# Autodesk Inventor assembly: plotter
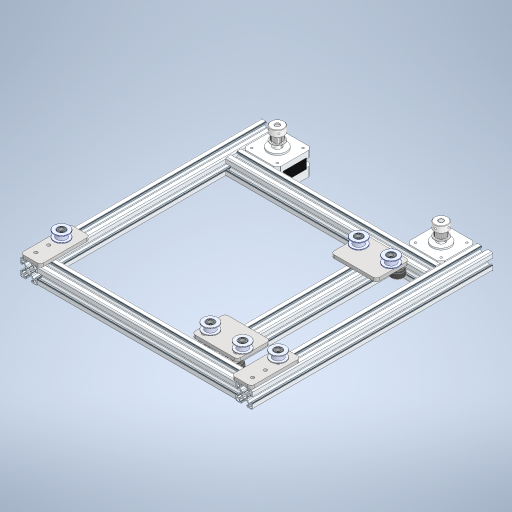
[picture p0: Inventor's stored thumbnail of the model, 512x512]
Saved by Autodesk Inventor 2023.1 (Build 271208000, 208)
## iProperties
Created: 2025-11-24
Part Number: plotter
Document SubType Name: Assembly
Designer: DELL
Author: DELL
## Documents named in this file (21)
- C:\Users\DELL\reposGitHub\VSOSH25-26\models\plotter\plotter.iam
- C:\Users\DELL\reposGitHub\VSOSH25-26\models\plotter\эскиз.ipt
- C:\Users\DELL\reposGitHub\VSOSH25-26\models\import\222LX-Konstruktsionnyy-profil-20kh20L.ipt
- C:\Users\DELL\reposGitHub\VSOSH25-26\models\plotter\профиль2020.ipt
- C:\Users\DELL\reposGitHub\VSOSH25-26\models\plotter\креп_мотора.ipt
- C:\Users\DELL\reposGitHub\VSOSH25-26\models\plotter\креп_мотора_MIR.ipt
- C:\Users\DELL\reposGitHub\VSOSH25-26\models\import\profil.ipt
- C:\Users\DELL\reposGitHub\VSOSH25-26\models\plotter\креп_центр_рейки.ipt
- C:\Users\DELL\reposGitHub\VSOSH25-26\models\import\Ролик с резьбой GT2 на моторы.ipt
- C:\Users\DELL\reposGitHub\VSOSH25-26\models\import\Сборка ролик с подшипником.ipt
- C:\Users\DELL\reposGitHub\VSOSH25-26\models\import\Ролик с резьбой GT2 на моторы_MIR.ipt
- C:\Users\DELL\reposGitHub\VSOSH25-26\models\import\Сборка ролик с подшипником_MIR1.ipt
- C:\Users\DELL\reposGitHub\VSOSH25-26\models\plotter\креп. пасс. ролика_MIR.ipt
- C:\Users\DELL\reposGitHub\VSOSH25-26\models\import\Stepper motor Nema 17 (17HS2408).ipt
- C:\Users\DELL\reposGitHub\VSOSH25-26\models\import\A177-Mini-plastikovyy-rolik-dlya-V_paza.ipt
- C:\Users\DELL\reposGitHub\VSOSH25-26\models\import\A183-Podshipnik-dlya-mini-rolikov_-_-5-_-10_-MR105zz.ipt
- C:\Users\DELL\reposGitHub\VSOSH25-26\models\plotter\креп_центр_рейки_MIR2.ipt
- C:\Users\DELL\reposGitHub\VSOSH25-26\models\import\Сборка ролик с подшипником_MIR2.ipt
- C:\Users\DELL\reposGitHub\VSOSH25-26\models\import\A177-Mini-plastikovyy-rolik-dlya-V_paza_MIR.ipt
- C:\Users\DELL\reposGitHub\VSOSH25-26\models\import\A183-Podshipnik-dlya-mini-rolikov_-_-5-_-10_-MR105zz_MIR.ipt
- C:\Users\DELL\reposGitHub\VSOSH25-26\models\import\original_prifil.ipt
## Components (35 placed, 22 different names)
1. эскиз:1
2. профиль24Левый — Совмещение:10, Заподлицо:2, Совмещение:12, Заподлицо:3, Совмещение:13, Совмещение:15, Совмещение:16, Совмещение:19, Совмещение:28, Совмещение:132, Касательность:8, Заподлицо:35, Касательность:9, Заподлицо:36
3. профиль16Верх:1 — Заподлицо:2, Совмещение:12, Совмещение:15, Совмещение:20, Совмещение:134, Заподлицо:37, Заподлицо:38, Совмещение:137
4. профиь26низ — Заподлицо:3, Совмещение:13, Совмещение:16, Заподлицо:27, Совмещение:102, Заподлицо:28, Совмещение:135, Заподлицо:39, Заподлицо:40, Заподлицо:43
5. креп_мотора:1
6. креп_мотора_MIR:1
7. profil:1 — Совмещение:25, Совмещение:28, Заподлицо:29, Совмещение:108, Заподлицо:34, Совмещение:133
8. креп_центр_рейки:1 — Заподлицо:29, Совмещение:108, Совмещение:110, Совмещение:111, Совмещение:113, Совмещение:115, Совмещение:116, Совмещение:117, Совмещение:118, Совмещение:119
9. Ролик с резьбой GT2 на моторы:1 — Совмещение:72
10. Сборка ролик с подшипником:1 — Совмещение:113, Совмещение:116, Совмещение:117
11. Сборка ролик с подшипником:2 — Совмещение:115, Совмещение:118, Совмещение:119
12. Сборка ролик с подшипником:3 — Совмещение:103, Совмещение:104
13. Ролик с резьбой GT2 на моторы_MIR:1 — Совмещение:105, Совмещение:106
14. креп. пасс. ролика_MIR:1 — Совмещение:68, Совмещение:69
15. Сборка ролик с подшипником_MIR1:3 — Совмещение:68, Совмещение:69
16. Stepper motor Nema 17 (17HS2408):1 — Совмещение:72, Совмещение:135, Заподлицо:39, Заподлицо:40, Совмещение:136, Заподлицо:42
17. Stepper motor Nema 17 (17HS2408):2 — Совмещение:105, Совмещение:106, Совмещение:134, Заподлицо:37, Заподлицо:38, Заподлицо:41, Совмещение:138
18. A177-Mini-plastikovyy-rolik-dlya-V_paza:3
19. A183-Podshipnik-dlya-mini-rolikov_-_-5-_-10_-MR105zz:5 — Совмещение:107
20. A183-Podshipnik-dlya-mini-rolikov_-_-5-_-10_-MR105zz:6 — Совмещение:107, Совмещение:110
21. A177-Mini-plastikovyy-rolik-dlya-V_paza:4
22. A183-Podshipnik-dlya-mini-rolikov_-_-5-_-10_-MR105zz:7
23. A183-Podshipnik-dlya-mini-rolikov_-_-5-_-10_-MR105zz:8 — Совмещение:111
24. креп. пасс. ролика_MIR:2 — Заподлицо:27, Совмещение:102, Заподлицо:28, Совмещение:103, Совмещение:104
25. креп_центр_рейки_MIR2:1 — Совмещение:120, Совмещение:121, Совмещение:122, Совмещение:123, Совмещение:124, Совмещение:125, Совмещение:126, Совмещение:130, Заподлицо:34, Совмещение:132, Совмещение:133
26. Сборка ролик с подшипником_MIR2:1 — Совмещение:120, Совмещение:121, Совмещение:122
27. Сборка ролик с подшипником_MIR2:2 — Совмещение:123, Совмещение:124, Совмещение:125
28. A177-Mini-plastikovyy-rolik-dlya-V_paza_MIR:1 — Заподлицо:30, Заподлицо:31, Совмещение:128, Касательность:8, Заподлицо:35
29. A183-Podshipnik-dlya-mini-rolikov_-_-5-_-10_-MR105zz_MIR:1 — Заподлицо:30, Совмещение:127
30. A183-Podshipnik-dlya-mini-rolikov_-_-5-_-10_-MR105zz_MIR:2 — Совмещение:126, Совмещение:127, Заподлицо:31, Совмещение:128
31. A177-Mini-plastikovyy-rolik-dlya-V_paza_MIR:2 — Заподлицо:32, Совмещение:129, Заподлицо:33, Совмещение:131, Касательность:9, Заподлицо:36
32. A183-Podshipnik-dlya-mini-rolikov_-_-5-_-10_-MR105zz_MIR:3 — Заподлицо:32, Совмещение:129
33. A183-Podshipnik-dlya-mini-rolikov_-_-5-_-10_-MR105zz_MIR:4 — Совмещение:130, Заподлицо:33, Совмещение:131
34. original_prifil:1 — Заподлицо:41, Совмещение:136, Заподлицо:42
35. 222LX-Konstruktsionnyy-profil-20kh20L:2 — Заподлицо:43, Совмещение:137, Совмещение:138
## Relationships (74: Mate 49, Flush 23, Tangent 2)
- Совмещение:10 [Mate]: профиль24Левый
- Заподлицо:2 [Flush]: профиль24Левый ↔ профиль16Верх:1
- Совмещение:12 [Mate]: профиль24Левый ↔ профиль16Верх:1
- Заподлицо:3 [Flush]: профиль24Левый ↔ профиь26низ
- Совмещение:13 [Mate]: профиль24Левый ↔ профиь26низ
- Совмещение:15 [Mate]: профиль24Левый ↔ профиль16Верх:1
- Совмещение:16 [Mate]: профиль24Левый ↔ профиь26низ
- Совмещение:19 [Mate] (110 mm): профиль24Левый
- Совмещение:20 [Mate] (120 mm): профиль16Верх:1
- Совмещение:25 [Mate]: profil:1
- Совмещение:28 [Mate] (5 mm): профиль24Левый ↔ profil:1
- Совмещение:68 [Mate]: креп. пасс. ролика_MIR:1 ↔ Сборка ролик с подшипником_MIR1:3
- Совмещение:69 [Mate] (5 mm): креп. пасс. ролика_MIR:1 ↔ Сборка ролик с подшипником_MIR1:3
- Совмещение:72 [Mate]: Ролик с резьбой GT2 на моторы:1 ↔ Stepper motor Nema 17 (17HS2408):1
- [Flush]: A177-Mini-plastikovyy-rolik-dlya-V_paza:3 ↔ A183-Podshipnik-dlya-mini-rolikov_-_-5-_-10_-MR105zz:5
- [Mate]: A177-Mini-plastikovyy-rolik-dlya-V_paza:3 ↔ A183-Podshipnik-dlya-mini-rolikov_-_-5-_-10_-MR105zz:6
- [Flush]: A177-Mini-plastikovyy-rolik-dlya-V_paza:3 ↔ A183-Podshipnik-dlya-mini-rolikov_-_-5-_-10_-MR105zz:6
- [Mate]: A177-Mini-plastikovyy-rolik-dlya-V_paza:4 ↔ A183-Podshipnik-dlya-mini-rolikov_-_-5-_-10_-MR105zz:7
- [Flush]: A177-Mini-plastikovyy-rolik-dlya-V_paza:4 ↔ A183-Podshipnik-dlya-mini-rolikov_-_-5-_-10_-MR105zz:7
- [Mate]: A177-Mini-plastikovyy-rolik-dlya-V_paza:4 ↔ A183-Podshipnik-dlya-mini-rolikov_-_-5-_-10_-MR105zz:8
- [Flush]: A177-Mini-plastikovyy-rolik-dlya-V_paza:4 ↔ A183-Podshipnik-dlya-mini-rolikov_-_-5-_-10_-MR105zz:8
- Заподлицо:27 [Flush]: профиь26низ ↔ креп. пасс. ролика_MIR:2
- Совмещение:102 [Mate]: профиь26низ ↔ креп. пасс. ролика_MIR:2
- Заподлицо:28 [Flush]: профиь26низ ↔ креп. пасс. ролика_MIR:2
- Совмещение:103 [Mate]: Сборка ролик с подшипником:3 ↔ креп. пасс. ролика_MIR:2
- Совмещение:104 [Mate]: Сборка ролик с подшипником:3 ↔ креп. пасс. ролика_MIR:2
- Совмещение:105 [Mate]: Ролик с резьбой GT2 на моторы_MIR:1 ↔ Stepper motor Nema 17 (17HS2408):2
- Совмещение:106 [Mate] (5 mm): Ролик с резьбой GT2 на моторы_MIR:1 ↔ Stepper motor Nema 17 (17HS2408):2
- Совмещение:107 [Mate]: A183-Podshipnik-dlya-mini-rolikov_-_-5-_-10_-MR105zz:5 ↔ A183-Podshipnik-dlya-mini-rolikov_-_-5-_-10_-MR105zz:6
- Заподлицо:29 [Flush] (-17.5 mm): profil:1 ↔ креп_центр_рейки:1
- Совмещение:108 [Mate]: profil:1 ↔ креп_центр_рейки:1
- Совмещение:110 [Mate]: креп_центр_рейки:1 ↔ A183-Podshipnik-dlya-mini-rolikov_-_-5-_-10_-MR105zz:6
- Совмещение:111 [Mate]: креп_центр_рейки:1 ↔ A183-Podshipnik-dlya-mini-rolikov_-_-5-_-10_-MR105zz:8
- Совмещение:113 [Mate]: креп_центр_рейки:1 ↔ Сборка ролик с подшипником:1
- Совмещение:115 [Mate]: креп_центр_рейки:1 ↔ Сборка ролик с подшипником:2
- Совмещение:116 [Mate]: креп_центр_рейки:1 ↔ Сборка ролик с подшипником:1
- Совмещение:117 [Mate]: креп_центр_рейки:1 ↔ Сборка ролик с подшипником:1
- Совмещение:118 [Mate]: креп_центр_рейки:1 ↔ Сборка ролик с подшипником:2
- Совмещение:119 [Mate]: креп_центр_рейки:1 ↔ Сборка ролик с подшипником:2
- Совмещение:120 [Mate]: креп_центр_рейки_MIR2:1 ↔ Сборка ролик с подшипником_MIR2:1
- Совмещение:121 [Mate]: креп_центр_рейки_MIR2:1 ↔ Сборка ролик с подшипником_MIR2:1
- Совмещение:122 [Mate]: креп_центр_рейки_MIR2:1 ↔ Сборка ролик с подшипником_MIR2:1
- Совмещение:123 [Mate]: креп_центр_рейки_MIR2:1 ↔ Сборка ролик с подшипником_MIR2:2
- Совмещение:124 [Mate]: креп_центр_рейки_MIR2:1 ↔ Сборка ролик с подшипником_MIR2:2
- Совмещение:125 [Mate]: креп_центр_рейки_MIR2:1 ↔ Сборка ролик с подшипником_MIR2:2
- Заподлицо:30 [Flush]: A177-Mini-plastikovyy-rolik-dlya-V_paza_MIR:1 ↔ A183-Podshipnik-dlya-mini-rolikov_-_-5-_-10_-MR105zz_MIR:1
- Совмещение:126 [Mate]: креп_центр_рейки_MIR2:1 ↔ A183-Podshipnik-dlya-mini-rolikov_-_-5-_-10_-MR105zz_MIR:2
- Совмещение:127 [Mate]: A183-Podshipnik-dlya-mini-rolikov_-_-5-_-10_-MR105zz_MIR:1 ↔ A183-Podshipnik-dlya-mini-rolikov_-_-5-_-10_-MR105zz_MIR:2
- Заподлицо:31 [Flush]: A177-Mini-plastikovyy-rolik-dlya-V_paza_MIR:1 ↔ A183-Podshipnik-dlya-mini-rolikov_-_-5-_-10_-MR105zz_MIR:2
- Совмещение:128 [Mate]: A177-Mini-plastikovyy-rolik-dlya-V_paza_MIR:1 ↔ A183-Podshipnik-dlya-mini-rolikov_-_-5-_-10_-MR105zz_MIR:2
- Заподлицо:32 [Flush]: A177-Mini-plastikovyy-rolik-dlya-V_paza_MIR:2 ↔ A183-Podshipnik-dlya-mini-rolikov_-_-5-_-10_-MR105zz_MIR:3
- Совмещение:129 [Mate]: A177-Mini-plastikovyy-rolik-dlya-V_paza_MIR:2 ↔ A183-Podshipnik-dlya-mini-rolikov_-_-5-_-10_-MR105zz_MIR:3
- Совмещение:130 [Mate]: креп_центр_рейки_MIR2:1 ↔ A183-Podshipnik-dlya-mini-rolikov_-_-5-_-10_-MR105zz_MIR:4
- Заподлицо:33 [Flush]: A177-Mini-plastikovyy-rolik-dlya-V_paza_MIR:2 ↔ A183-Podshipnik-dlya-mini-rolikov_-_-5-_-10_-MR105zz_MIR:4
- Совмещение:131 [Mate]: A177-Mini-plastikovyy-rolik-dlya-V_paza_MIR:2 ↔ A183-Podshipnik-dlya-mini-rolikov_-_-5-_-10_-MR105zz_MIR:4
- Заподлицо:34 [Flush] (17.5 mm): profil:1 ↔ креп_центр_рейки_MIR2:1
- Совмещение:132 [Mate]: профиль24Левый ↔ креп_центр_рейки_MIR2:1
- Совмещение:133 [Mate]: profil:1 ↔ креп_центр_рейки_MIR2:1
- Касательность:8 [Tangent] (-0.9 mm): профиль24Левый ↔ A177-Mini-plastikovyy-rolik-dlya-V_paza_MIR:1
- Заподлицо:35 [Flush] (5.6 mm): профиль24Левый ↔ A177-Mini-plastikovyy-rolik-dlya-V_paza_MIR:1
- Касательность:9 [Tangent] (-0.9 mm): профиль24Левый ↔ A177-Mini-plastikovyy-rolik-dlya-V_paza_MIR:2
- Заподлицо:36 [Flush] (5.6 mm): профиль24Левый ↔ A177-Mini-plastikovyy-rolik-dlya-V_paza_MIR:2
- Совмещение:134 [Mate]: профиль16Верх:1 ↔ Stepper motor Nema 17 (17HS2408):2
- Заподлицо:37 [Flush]: профиль16Верх:1 ↔ Stepper motor Nema 17 (17HS2408):2
- Заподлицо:38 [Flush]: профиль16Верх:1 ↔ Stepper motor Nema 17 (17HS2408):2
- Совмещение:135 [Mate]: профиь26низ ↔ Stepper motor Nema 17 (17HS2408):1
- Заподлицо:39 [Flush]: профиь26низ ↔ Stepper motor Nema 17 (17HS2408):1
- Заподлицо:40 [Flush]: профиь26низ ↔ Stepper motor Nema 17 (17HS2408):1
- Заподлицо:41 [Flush]: Stepper motor Nema 17 (17HS2408):2 ↔ original_prifil:1
- Совмещение:136 [Mate]: Stepper motor Nema 17 (17HS2408):1 ↔ original_prifil:1
- Заподлицо:42 [Flush]: Stepper motor Nema 17 (17HS2408):1 ↔ original_prifil:1
- Заподлицо:43 [Flush]: профиь26низ ↔ 222LX-Konstruktsionnyy-profil-20kh20L:2
- Совмещение:137 [Mate]: профиль16Верх:1 ↔ 222LX-Konstruktsionnyy-profil-20kh20L:2
- Совмещение:138 [Mate]: Stepper motor Nema 17 (17HS2408):2 ↔ 222LX-Konstruktsionnyy-profil-20kh20L:2
## Named parameters: d136_d130 = 0 mm, d137_d131 = 0 mm, d138_d132 = 0 mm, d141_d135_d129 = 0 mm, d142_d136_d130 = 0 mm, d143_d137_d131 = 0 mm, d144_d138_d132 = 0 mm
